# Autodesk Inventor assembly: F_TOPO
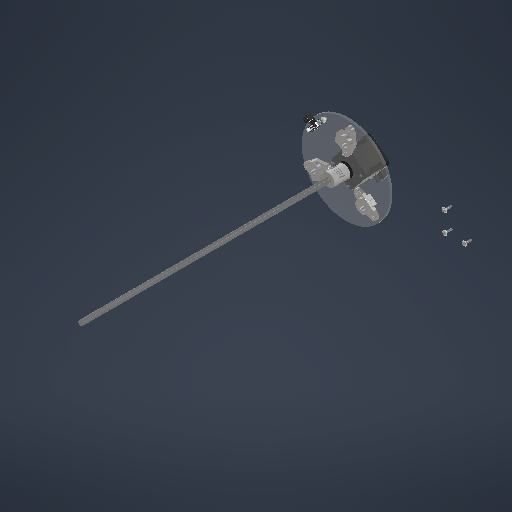
[picture p0: Inventor's stored thumbnail of the model, 512x512]
Saved by Autodesk Inventor 2025.2 (Build 292293000, 293)
## iProperties
Created: 2025-05-02
Part Number: F_TOPO
Document SubType Name: Assembly
Designer: Nelson
Author: Nelson
## Documents named in this file (10)
- C:\Users\Tiago\Documents\Inventor\Exp. Braço v1\F_TOPO.iam
- C:\Users\Tiago\Documents\Inventor\Exp. Braço v1\Topo.ipt
- C:\Users\Tiago\Documents\Inventor\Exp. Braço v1\Lead screw 2pitch_8lead_400mm.ipt
- C:\Users\Tiago\Documents\Inventor\Exp. Braço v1\NEMA17 42-38.ipt
- C:\Users\Tiago\Documents\Inventor\Exp. Braço v1\shaft_coupler 5mm_to_8mm.ipt
- C:\Users\Tiago\Documents\Inventor\Exp. Braço v1\Linear_Shaft_Support_SHF10.ipt
- C:\Users\Tiago\Documents\Inventor\Exp. Braço v1\Limit_Switch.ipt
- C:\Users\Tiago\Documents\Inventor\Exp. Braço v1\Anilha_M3.ipt
- C:\Users\Tiago\Documents\Inventor\Exp. Braço v1\M3 x0.5 ALT (...).ipt
- C:\Users\Tiago\Documents\Inventor\Exp. Braço v1\Porca_sextavada(3M).ipt
## Components (20 placed, 9 different names)
1. Topo:1 — Mate:1, Mate:2, Mate:3, Mate:4, Mate:5, Mate:6, Mate:7, Mate:8, Mate:9, Mate:10, Mate:11, Mate:12, Mate:17, Mate:18, Mate:19, Insert:1, Insert:4, Insert:6, Insert:8, Mate:22, Mate:23, Mate:24
2. Lead screw 2pitch_8lead_400mm:1 — Mate:13, Mate:14, Mate:16, Rotation:1
3. NEMA17 42-38:1 — Mate:2, Mate:3, Mate:14, Mate:15, Mate:16, Mate:24
4. shaft_coupler 5mm_to_8mm:1 — Mate:13, Mate:15, Rotation:1
5. Linear_Shaft_Support_SHF10:1 — Mate:4, Mate:9, Mate:10
6. Linear_Shaft_Support_SHF10:2 — Mate:5, Mate:7, Mate:12
7. Linear_Shaft_Support_SHF10:3 — Mate:6, Mate:8, Mate:11
8. Limit_Switch:1 — Mate:17, Mate:18, Mate:19, Insert:9, Insert:10
9. Anilha_M3:1 — Insert:1, Insert:2
10. M3 x0.5 ALT (...):1 — Insert:2
11. Anilha_M3:2 — Insert:4
12. M3 x0.5 ALT (...):2
13. Anilha_M3:3 — Insert:6
14. M3 x0.5 ALT (...):3
15. Anilha_M3:4 — Insert:8
16. M3 x0.5 ALT (...):4
17. M3 x0.5 ALT (...):5 — Insert:9, Mate:20
18. M3 x0.5 ALT (...):6 — Insert:10, Mate:21
19. Porca_sextavada(3M):1 — Mate:21, Mate:22
20. Porca_sextavada(3M):2 — Mate:20, Mate:23
## Relationships (35: Mate 24, Insert 10, RelateRotation 1)
- Mate:1: Topo:1
- Mate:2: Topo:1 ↔ NEMA17 42-38:1
- Mate:3: Topo:1 ↔ NEMA17 42-38:1
- Mate:4: Topo:1 ↔ Linear_Shaft_Support_SHF10:1
- Mate:5: Topo:1 ↔ Linear_Shaft_Support_SHF10:2
- Mate:6: Topo:1 ↔ Linear_Shaft_Support_SHF10:3
- Mate:7: Topo:1 ↔ Linear_Shaft_Support_SHF10:2
- Mate:8: Topo:1 ↔ Linear_Shaft_Support_SHF10:3
- Mate:9: Topo:1 ↔ Linear_Shaft_Support_SHF10:1
- Mate:10: Topo:1 ↔ Linear_Shaft_Support_SHF10:1
- Mate:11: Topo:1 ↔ Linear_Shaft_Support_SHF10:3
- Mate:12: Topo:1 ↔ Linear_Shaft_Support_SHF10:2
- Mate:13: Lead screw 2pitch_8lead_400mm:1 ↔ shaft_coupler 5mm_to_8mm:1
- Mate:14: Lead screw 2pitch_8lead_400mm:1 ↔ NEMA17 42-38:1
- Mate:15 (5 mm): NEMA17 42-38:1 ↔ shaft_coupler 5mm_to_8mm:1
- Mate:16 (1 mm): Lead screw 2pitch_8lead_400mm:1 ↔ NEMA17 42-38:1
- Mate:17: Topo:1 ↔ Limit_Switch:1
- Mate:18: Topo:1 ↔ Limit_Switch:1
- Mate:19: Topo:1 ↔ Limit_Switch:1
- Rotation:1 [RelateRotation] (1 ul): Lead screw 2pitch_8lead_400mm:1 ↔ shaft_coupler 5mm_to_8mm:1
- Insert:1: Topo:1 ↔ Anilha_M3:1
- Insert:2: Anilha_M3:1 ↔ M3 x0.5 ALT (...):1
- [Insert]: Anilha_M3:2 ↔ M3 x0.5 ALT (...):2
- Insert:4: Topo:1 ↔ Anilha_M3:2
- [Insert]: Anilha_M3:3 ↔ M3 x0.5 ALT (...):3
- Insert:6: Topo:1 ↔ Anilha_M3:3
- [Insert]: Anilha_M3:4 ↔ M3 x0.5 ALT (...):4
- Insert:8: Topo:1 ↔ Anilha_M3:4
- Insert:9: Limit_Switch:1 ↔ M3 x0.5 ALT (...):5
- Insert:10: Limit_Switch:1 ↔ M3 x0.5 ALT (...):6
- Mate:20: M3 x0.5 ALT (...):5 ↔ Porca_sextavada(3M):2
- Mate:21: M3 x0.5 ALT (...):6 ↔ Porca_sextavada(3M):1
- Mate:22: Topo:1 ↔ Porca_sextavada(3M):1
- Mate:23: Topo:1 ↔ Porca_sextavada(3M):2
- Mate:24: Topo:1 ↔ NEMA17 42-38:1
## Named parameters: d23_d22 = 0 mm, d25_d22 = 0 mm, d27_d22 = 0 mm
